# Autodesk Inventor assembly: Camera Mount
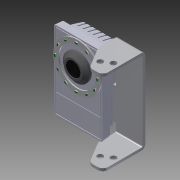
[picture p0: Inventor's stored thumbnail of the model, 180x180]
Saved by Autodesk Inventor 2014 SP1 (Build 180222100, 222)
## iProperties
Created: 2012-03-02
Part Number: Camera Mount
Document SubType Name: Assembly
Designer: Moses
Mass: 164.178 g
Surface Area: 370.907 cm^2
Volume: 127.605 cm^3
Density: 1.28661 g/cm^3
Author: Moses
## Documents named in this file (5)
- C:\Users\Moses\Documents\Inventor\Rebuild\Repackaged_Team 3061_2012 Ball Shooter_Inventor Version_2014\Camera Mount.iam
- C:\Users\Moses\Documents\Inventor\Rebuild\Repackaged_Team 3061_2012 Ball Shooter_Inventor Version_2014\AXIS-M1011.ipt
- C:\Users\Moses\Documents\Inventor\Rebuild\Repackaged_Team 3061_2012 Ball Shooter_Inventor Version_2014\Camera Bracket.ipt
- C:\Users\Moses\Documents\Inventor\Rebuild\Repackaged_Team 3061_2012 Ball Shooter_Inventor Version_2014\IFI 100_107 - No. 6 - 32 Metal Type.ipt
- C:\Users\Moses\Documents\Inventor\Rebuild\Repackaged_Team 3061_2012 Ball Shooter_Inventor Version_2014\LED Ring.ipt
## Components (4 placed, 4 different names)
1. AXIS-M1011:1 — Mate:1, Mate:2, Angle:1, Insert:2
2. Camera Bracket:1 — Mate:1, Mate:2, Angle:1, Insert:1
3. Prevailing Torque Type Hex Nut - Inch (IFI) No. 6 - 32 Metal Type:1 — Insert:1
4. LED Ring:1 — Insert:2
## Relationships (5: Mate 2, Insert 2, Angle 1)
- Mate:1: AXIS-M1011:1 ↔ Camera Bracket:1
- Mate:2: AXIS-M1011:1 ↔ Camera Bracket:1
- Angle:1 (180 deg): AXIS-M1011:1 ↔ Camera Bracket:1
- Insert:1: Camera Bracket:1 ↔ Prevailing Torque Type Hex Nut - Inch (IFI) No. 6 - 32 Metal Type:1
- Insert:2: AXIS-M1011:1 ↔ LED Ring:1
